# Autodesk Inventor assembly: 217-3141-RS775-STEP
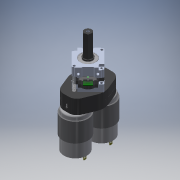
[picture p0: Inventor's stored thumbnail of the model, 180x180]
Saved by Autodesk Inventor 2018 (Build 220112000, 112)
## iProperties
Created: 2014-01-14
Part Number: 217-3141-RS775-STEP
Description: STEP AP214
Document SubType Name: Assembly
Designer: snipe
Sending System: SolidWorks 2013
Preprocessor: SwSTEP 2.0
Title: 217-3141-RS775-STEP.STEP
Revision Number: ANY
## Documents named in this file (15)
- E:\50000skater\Assets\VPlan775dualinput.iam
- E:\50000skater\Assets\Resources\217-3141-001 Rev1.ipt
- E:\50000skater\Assets\Resources\217-3141-007 Rev1_30T 32DP.ipt
- E:\50000skater\Assets\Resources\217-3141-006 Rev1_30T 32DP.ipt
- E:\50000skater\Assets\Resources\217-2741.ipt
- E:\50000skater\Assets\Resources\PINL-M020-006-S.ipt
- E:\50000skater\Assets\Resources\SSS1032-0188-ZB.ipt
- E:\50000skater\Assets\Resources\NUT-832-NYLOCK.ipt
- E:\50000skater\Assets\Resources\91251A346_91251A346.ipt
- E:\50000skater\Assets\Resources\SSA_SSAM4-0010ZC.ipt
- E:\50000skater\Assets\Resources\SSA_SSA0832-0750ZC.ipt
- E:\50000skater\Assets\Resources\217-3141-004 Rev1.ipt
- E:\50000skater\Assets\Resources\BB RS775-18V.ipt
- E:\50000skater\Assets\Resources\217-2625-013 Rev1.ipt
- E:\50000skater\Assets\VPlanRingGear.iam
## Components (25 placed, 25 different names)
1. 217-3141-001 Rev1_1 — Mate:3
2. 217-3141-007 Rev1_30T 32DP_2 — Mate:1
3. 217-3141-006 Rev1_30T 32DP_3
4. 217-3141-006 Rev1_30T 32DP_4
5. 217-2741_5
6. 217-2741_6
7. PINL-M020-006-S_7
8. SSS1032-0188-ZB_8
9. SSS1032-0188-ZB_9
10. NUT-832-NYLOCK_10
11. NUT-832-NYLOCK_11
12. 91251A346_91251A346_12
13. 91251A346_91251A346_13 — Mate:2
14. SSA_SSAM4-0010ZC_14
15. SSA_SSA0832-0750ZC_15
16. SSA_SSA0832-0750ZC_16
17. SSA_SSAM4-0010ZC_17
18. SSA_SSAM4-0010ZC_18
19. SSA_SSAM4-0010ZC_19
20. 217-3141-004 Rev1_20
21. BB RS775-18V_21
22. BB RS775-18V_22
23. 217-2625-013 Rev1_23
24. 217-2625-013 Rev1_24
25. VPlanRingGear:1 [sub-assembly] — Mate:1, Mate:2, Mate:3
## Relationships (3: Mate 3)
- Mate:1: 217-3141-007 Rev1_30T 32DP_2 ↔ VPlanRingGear:1
- Mate:2: 91251A346_91251A346_13 ↔ VPlanRingGear:1
- Mate:3: 217-3141-001 Rev1_1 ↔ VPlanRingGear:1
